# Autodesk Inventor assembly: robot_2
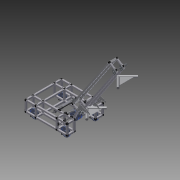
[picture p0: Inventor's stored thumbnail of the model, 180x180]
Saved by Autodesk Inventor 2011 (Build 150239000, 239)
## iProperties
Created: 2013-01-17
Part Number: robot_2
Document SubType Name: Assembly
Designer: Christopher
Author: Christopher
## Documents named in this file (8)
- F:\Users\Christopher\Documents\GitHub\2013CAD\2013 robot\forklift\robot_2.iam
- F:\Users\Christopher\Documents\GitHub\2013CAD\2013 robot\forklift\frame parts\forklift_1_0.iam
- F:\Users\Christopher\Documents\GitHub\2013CAD\2013 robot\forklift\robot_frame\frame_1_0.iam
- F:\Users\Christopher\Documents\GitHub\2013CAD\2013 robot\forklift\Pneumatics and frame grabbers\steadier_grabber.iam
- F:\Users\Christopher\Documents\GitHub\2013CAD\2013 robot\forklift\Pneumatics and frame grabbers\wheel_rider.iam
- F:\Users\Christopher\Documents\GitHub\2013CAD\2013 robot\forklift\Pneumatics and frame grabbers\cross_frame_axle.iam
- F:\Users\Christopher\Documents\GitHub\2013CAD\2013 robot\forklift\Pneumatics and frame grabbers\driving motors.iam
- F:\Users\Christopher\Documents\GitHub\2013CAD\2013 robot\forklift\Pneumatics and frame grabbers\wheel mount.iam
## Components (10 placed, 7 different names)
1. forklift_1_0:1 [sub-assembly] — Insert:4, Tangent:1
2. frame_1_0:1 [sub-assembly] — Insert:1, Insert:2, Insert:3, Flush:1, Mate:1, Mate:2, Mate:3, Flush:2, Flush:3, Mate:4, Flush:4, Mate:5, Flush:5, Flush:6, Mate:6, Flush:7, Flush:8, Mate:7, Flush:9, Flush:10, Mate:8, Flush:11, Flush:12
3. steadier_grabber:1 [sub-assembly] — Insert:1, Insert:2, Insert:3, Insert:4
4. wheel_rider:1 [sub-assembly] — Flush:1, Mate:1, Mate:2
5. cross_frame_axle:1 [sub-assembly] — Mate:3, Flush:2, Tangent:1
6. driving motors:1 [sub-assembly] — Flush:3, Mate:4, Flush:4
7. wheel mount:1 [sub-assembly] — Mate:5, Flush:5, Flush:6
8. wheel mount:2 [sub-assembly] — Mate:8, Flush:11, Flush:12
9. wheel mount:3 [sub-assembly] — Mate:6, Flush:7, Flush:8
10. wheel mount:4 [sub-assembly] — Mate:7, Flush:9, Flush:10
## Relationships (25: Flush 12, Mate 8, Insert 4, Tangent 1)
- Insert:1: frame_1_0:1 ↔ steadier_grabber:1
- Insert:2: frame_1_0:1 ↔ steadier_grabber:1
- Insert:3: frame_1_0:1 ↔ steadier_grabber:1
- Insert:4 (203.2 mm): forklift_1_0:1 ↔ steadier_grabber:1
- Flush:1 (6.35 mm): frame_1_0:1 ↔ wheel_rider:1
- Mate:1: frame_1_0:1 ↔ wheel_rider:1
- Mate:2 (50.8 mm): frame_1_0:1 ↔ wheel_rider:1
- Mate:3: frame_1_0:1 ↔ cross_frame_axle:1
- Flush:2: frame_1_0:1 ↔ cross_frame_axle:1
- Tangent:1: forklift_1_0:1 ↔ cross_frame_axle:1
- Flush:3: frame_1_0:1 ↔ driving motors:1
- Mate:4: frame_1_0:1 ↔ driving motors:1
- Flush:4 (152.4 mm): frame_1_0:1 ↔ driving motors:1
- Mate:5: frame_1_0:1 ↔ wheel mount:1
- Flush:5: frame_1_0:1 ↔ wheel mount:1
- Flush:6 (76.2 mm): frame_1_0:1 ↔ wheel mount:1
- Mate:6: frame_1_0:1 ↔ wheel mount:3
- Flush:7: frame_1_0:1 ↔ wheel mount:3
- Flush:8 (76.2 mm): frame_1_0:1 ↔ wheel mount:3
- Mate:7: frame_1_0:1 ↔ wheel mount:4
- Flush:9: frame_1_0:1 ↔ wheel mount:4
- Flush:10 (76.2 mm): frame_1_0:1 ↔ wheel mount:4
- Mate:8: frame_1_0:1 ↔ wheel mount:2
- Flush:11: frame_1_0:1 ↔ wheel mount:2
- Flush:12 (76.2 mm): frame_1_0:1 ↔ wheel mount:2
